# Autodesk Inventor assembly: Tenonfull
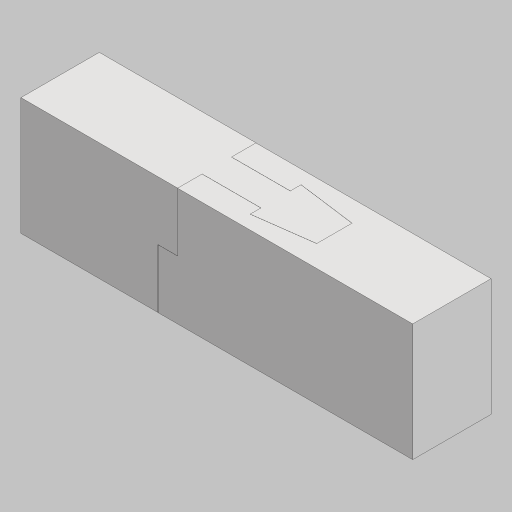
[picture p0: Inventor's stored thumbnail of the model, 512x512]
Saved by Autodesk Inventor 2023 (Build 270158000, 158)
## iProperties
Created: 2026-02-15
Part Number: Tenonfull
Document SubType Name: Assembly
Designer: MARTIN MAESTRE
Author: MARTIN MAESTRE
## Documents named in this file (3)
- C:\Users\MARTIN MAESTRE\OneDrive - Universidad de los Andes\POSTGRADO\202610\MAESTRIA\PROBLEMA ESPECIAL\CADS\Fig1\Tenonfull.iam
- C:\Users\MARTIN MAESTRE\OneDrive - Universidad de los Andes\POSTGRADO\202610\MAESTRIA\PROBLEMA ESPECIAL\CADS\Fig1\Tenon.ipt
- C:\Users\MARTIN MAESTRE\OneDrive - Universidad de los Andes\POSTGRADO\202610\MAESTRIA\PROBLEMA ESPECIAL\CADS\Fig1\Tenon2.ipt
## Components (2 placed, 2 different names)
1. Tenon:1 — Nivelación:1, Nivelación:2, Coincidencia:1, Coincidencia:2, Coincidencia:3
2. Tenon2:1 — Coincidencia:2, Coincidencia:3
## Relationships (5: Mate 3, Flush 2)
- Nivelación:1 [Flush]: Tenon:1
- Nivelación:2 [Flush]: Tenon:1
- Coincidencia:1 [Mate]: Tenon:1
- Coincidencia:2 [Mate]: Tenon:1 ↔ Tenon2:1
- Coincidencia:3 [Mate]: Tenon:1 ↔ Tenon2:1
